# Autodesk Inventor assembly: накладка
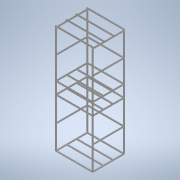
[picture p0: Inventor's stored thumbnail of the model, 180x180]
Saved by Autodesk Inventor 2020.1 (Build 241239000, 239)
## iProperties
Created: 2019-07-24
Part Number: накладка
Document SubType Name: Свариваемая деталь
Designer: Xardas
Weld Material: Сталь AISI 1050
Mass: 28824.2 g
Surface Area: 36847.5 cm^2
Volume: 3671.87 cm^3
Density: 7.85 g/cm^3
_SolveAssemblyDoc: Frame Generator Solve Assembly
_Version: 15.0.0
Author: Xardas
## Documents named in this file (3)
- E:\Work\Personal\3ds\2 этаж на стиралку - сварка\накладка.iam
- E:\Work\Personal\3ds\2 этаж на стиралку - сварка\Рама.ipt
- E:\Work\Personal\3ds\2 этаж на стиралку - сварка\Frame 1564003398286.iam
## Components (2 placed, 2 different names)
1. Рама:1 — Заподлицо:1
2. Frame 1564003398286:1 [sub-assembly]
## Relationships (1: Flush 1)
- Заподлицо:1 [Flush]: Рама:1
